# Autodesk Inventor assembly: Assembly_Kolbentank
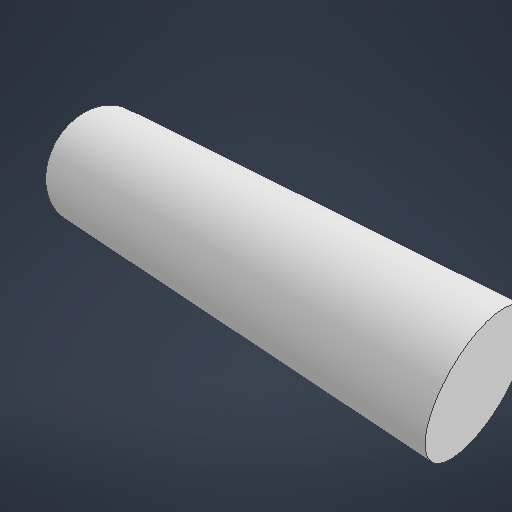
[picture p0: Inventor's stored thumbnail of the model, 512x512]
Saved by Autodesk Inventor 2026 (Build 300175000, 175)
## iProperties
Created: 2025-04-25
Part Number: Assembly_Kolbentank
Document SubType Name: Assembly
Designer: FAL
Author: FAL
## Documents named in this file (2)
- C:\Users\FAL\Projekte\Git\U-BERT\CAD\Kolbentank\Assembly_Kolbentank.iam
- C:\Users\FAL\Projekte\Git\U-BERT\CAD\Kolbentank\P_Spritze_60ml.ipt
## Components (1 placed, 1 different names)
1. P_Spritze_60ml:1 — Fluchtend:2, Fluchtend:3, Fluchtend:4
## Relationships (3: Flush 3)
- Fluchtend:2 [Flush]: P_Spritze_60ml:1
- Fluchtend:3 [Flush]: P_Spritze_60ml:1
- Fluchtend:4 [Flush]: P_Spritze_60ml:1
